# Autodesk Inventor assembly: SKF_7200 BECBP
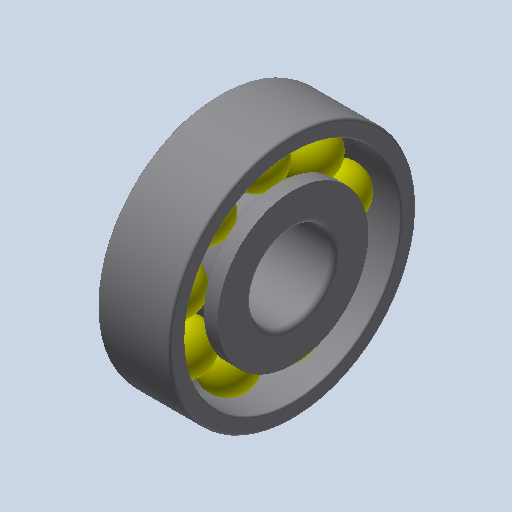
[picture p0: Inventor's stored thumbnail of the model, 512x512]
Saved by Autodesk Inventor 2022 (Build 260153000, 153)
## iProperties
Category: PARTsolutions
Company: SKF
Created: 2022-07-15
Part Number: SKF_7200 BECBP
Catalog Web Link: www.cadenas.de
Description: BA1_001_101-Angular contact ball bearings, single row
Vendor: SKF
Document SubType Name: Assembly
Designer: psAdmin
Manufacturer: SKF
Mass: 30 g
Surface Area: 40.6566 cm^2
Volume: 3.84326 cm^3
Density: 7.80587 g/cm^3
PSOL_IDENT_0: {$CADENAS_DATA/23d-libs/skf/bearings_units_and_housings/ball_bearings/angular_contact_ball_bearings/
PSOL_IDENT_1: ba1_001_101.prj},177 {VTYP=3D},{NB=SKF_7200 BECBP},{LINA=SKF_7200 BECBP},{NN=BA1_001_101},{DATE=08.0
PSOL_IDENT_2: 7.2022 10:24:26},{GEOMDATE=04.07.2022 06:53:14},{VERSION=},{LINEID=141430},{WBVAR=},{WBNUMERIC=}  {N
PSOL_IDENT_3: B=SKF_7200 BECBP},{LINA=SKF_7200 BECBP},{KT=DUMMY},{DESIGNATION=7200 BECBP},{DD=10.000},{D=30.000},{
PSOL_IDENT_4: B=9.0000},{DD1=18.300},{DD2=14.570},{D1=22.850},{D2=26.180},{D3=0.000},{D4=26.180},{D5=},{C1=0.000},
PSOL_IDENT_5: {AA=13},{R12=0.600},{R34=0.300},{ALPHA=40},{PITCH=20.300},{DW=6.000},{DDAMIN=14.2},{DDAMAX=},{DAMAX=
PSOL_IDENT_6: 25.8},{DBMAX=27.6},{RAMAX=0.6},{RBMAX=0.3},{LOAD1=7.02},{LOAD2=3.35},{LOAD3=0.14},{SPEED1=30000},{SP
PSOL_IDENT_7: EED2=30000},{Z=9},{II=1},{MASS=0.03},{BEARING=7200 BECBP},{POPULAR=Yes},{VARIANT=acbb1},{D2A=},{DD2A=
PSOL_IDENT_8: 14.570},{R5R=0.3},{R34L=0.6},{IRH=1},{ORH=1},{D4H=0.6}
NB: SKF_7200 BECBP
NN: BA1_001_101
NT: Angular contact ball bearings, single row
NBSYN: SKF_$DESIGNATION.
LINA: SKF_7200 BECBP
CATALOG: SKF
DESIGNATION: 7200 BECBP
DD: 10
D: 30
B: 9
LOAD1: 7.02
LOAD2: 3.35
LOAD3: 0.14
SPEED1: 30000
SPEED2: 30000
SUPPLIER: SKF
ARTICLENO: SKF_7200 BECBP
BOMINFO: SKF_7200 BECBP
CREATOR: CADENAS GmbH
Schulterdurchmesser_Ig: 18,300 mm
Schulterdurchmesser_Ik: 14,500 mm
Schulterdurchmesser_Ag: 22,800 mm
Title: SKF_7200 BECBP
Author: Cadenas PARTsolutions
Comments: Angular contact ball bearings, single row
## Documents named in this file (4)
- C:\Users\AEWALDER\Documents\Inventor\03_CurrentProjects\MasterThesis\PSM_V1_Rillenkugellager\SKF_7200 BECBP.iam
- C:\Users\AEWALDER\Documents\Inventor\03_CurrentProjects\MasterThesis\PSM_V1_Rillenkugellager\SKF_7200 BECBP_PART1.ipt
- C:\Users\AEWALDER\Documents\Inventor\03_CurrentProjects\MasterThesis\PSM_V1_Rillenkugellager\SKF_7200 BECBP_PART2.ipt
- C:\Users\AEWALDER\Documents\Inventor\03_CurrentProjects\MasterThesis\PSM_V1_Rillenkugellager\SKF_7200 BECBP_PART3.ipt
## Components (11 placed, 3 different names)
1. SKF_7200 BECBP_PART1:1
2. SKF_7200 BECBP_PART2:1
3. SKF_7200 BECBP_PART3:1
4. SKF_7200 BECBP_PART3:2
5. SKF_7200 BECBP_PART3:3
6. SKF_7200 BECBP_PART3:4
7. SKF_7200 BECBP_PART3:5
8. SKF_7200 BECBP_PART3:6
9. SKF_7200 BECBP_PART3:7
10. SKF_7200 BECBP_PART3:8
11. SKF_7200 BECBP_PART3:9
## Named parameters: Schulterdurchmesser_Ig = 18.3 mm, Schulterdurchmesser_Ik = 14.5 mm, Schulterdurchmesser_Ag = 22.8 mm
